# Autodesk Inventor assembly: SPE0V1 Ensamble General
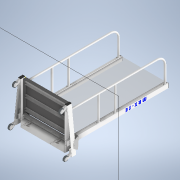
[picture p0: Inventor's stored thumbnail of the model, 180x180]
Saved by Autodesk Inventor 2021.2 (Build 252289000, 289)
## iProperties
Created: 2026-05-12
Part Number: SPE0V1 Ensamble General
Document SubType Name: Assembly
Designer: nelso
Author: nelso
## Documents named in this file (14)
- C:\Users\nelso\Desktop\Soporte-Paciente-Espinografia\Workspace\SPE0V1 Ensamble General.iam
- C:\Users\nelso\Desktop\Soporte-Paciente-Espinografia\Workspace\SP25V1 Acrilico.ipt
- C:\Users\nelso\Desktop\Soporte-Paciente-Espinografia\Workspace\SPE1V1 Estructura.iam
- C:\Users\nelso\Desktop\Soporte-Paciente-Espinografia\Workspace\SPE2V1 Baranda.iam
- C:\Users\nelso\Desktop\Soporte-Paciente-Espinografia\Workspace\DIN933M8X1.25L20C.ipt
- C:\Users\nelso\Desktop\Soporte-Paciente-Espinografia\Workspace\DIN125-A8,4C.ipt
- C:\Users\nelso\Desktop\Soporte-Paciente-Espinografia\Workspace\Logo.ipt
- C:\Users\nelso\Desktop\Soporte-Paciente-Espinografia\Workspace\SP28V1 Seguro Acrilico.ipt
- C:\Users\nelso\Desktop\Soporte-Paciente-Espinografia\Workspace\SP26V1 Base Chapa.ipt
- C:\Users\nelso\Desktop\Soporte-Paciente-Espinografia\Workspace\SP32V1 Refuerzo.ipt
- C:\Users\nelso\Desktop\Soporte-Paciente-Espinografia\Workspace\SPE31V1 Bisagra.iam
- C:\Users\nelso\Desktop\Soporte-Paciente-Espinografia\Workspace\SP39V1 Chapa Acrilico.ipt
- C:\Users\nelso\Desktop\Soporte-Paciente-Espinografia\Workspace\ISO7380M4X0.8L16I.ipt
- C:\Users\nelso\Desktop\Soporte-Paciente-Espinografia\Workspace\DIN555-5M4X0.8I.ipt
## Components (84 placed, 13 different names)
1. SP26V1 Base Chapa:1 — Mate:343, Mate:344, Mate:345, Mate:346, Mate:347, Mate:348, Mate:350, Mate:351, Mate:352, Mate:353, Mate:354, Flush:49, Flush:50, Flush:51, Angle:1
2. SP25V1 Acrilico:1 — Mate:179, Mate:180, Flush:19, Flush:20, Mate:262, Mate:355, Mate:356, Mate:357, Flush:52, Flush:53
3. SPE1V1 Estructura:1 [sub-assembly] — Coincidencia:100, Coincidencia:101, Coincidencia:102, Coincidencia:117, Nivelación:14, Nivelación:15, Mate:235, Mate:236, Mate:237, Flush:40, Mate:239, Mate:240, Mate:241, Flush:42, Mate:324, Mate:325, Flush:47, Flush:48, Mate:331, Mate:332, Mate:333, Mate:337, Mate:338, Mate:339, Mate:340, Mate:341, Mate:342, Angle:1, Flush:52
4. SPE2V1 Baranda:2 [sub-assembly] — Coincidencia:100, Coincidencia:101, Coincidencia:102, Coincidencia:109, Coincidencia:110, Coincidencia:111, Coincidencia:112, Mate:134, Mate:135, Mate:136, Mate:137, Mate:138, Mate:139, Mate:140, Mate:141, Mate:142, Mate:143, Mate:144, Mate:145, Mate:168, Mate:169, Mate:170, Mate:171, Mate:172, Mate:173
5. SPE2V1 Baranda:3 [sub-assembly] — Mate:118, Mate:119, Mate:120, Mate:121, Mate:122, Mate:123, Mate:124, Mate:125, Mate:126, Mate:127, Mate:128, Mate:129, Mate:130, Mate:131, Mate:132, Mate:133, Mate:147, Mate:149, Mate:156, Mate:157, Mate:158, Mate:159, Mate:160, Mate:161, Mate:235, Mate:236
6. DIN933M8X1.25L20C:1 — Coincidencia:113, Coincidencia:114
7. DIN125-A8,4C:1 — Coincidencia:109, Coincidencia:110, Coincidencia:115, Coincidencia:116
8. DIN125-A8,4C:2 — Coincidencia:111, Coincidencia:112, Coincidencia:113, Coincidencia:114
9. DIN933M8X1.25L20C:2 — Coincidencia:115, Coincidencia:116
10. Logo:1 — Coincidencia:117, Nivelación:14, Nivelación:15
11. DIN125-A8,4C:3 — Mate:144, Mate:145, Mate:162
12. DIN125-A8,4C:4 — Mate:142, Mate:143, Mate:163
13. DIN125-A8,4C:5 — Mate:140, Mate:141, Mate:164
14. DIN125-A8,4C:6 — Mate:138, Mate:139, Mate:165
15. DIN125-A8,4C:7 — Mate:135, Mate:136, Mate:167
16. DIN125-A8,4C:8 — Mate:134, Mate:137, Mate:166
17. DIN125-A8,4C:9 — Mate:130, Mate:132, Mate:155
18. DIN125-A8,4C:10 — Mate:131, Mate:133, Mate:154
19. DIN125-A8,4C:11 — Mate:128, Mate:129, Mate:153
20. DIN125-A8,4C:12 — Mate:126, Mate:127, Mate:152
21. DIN125-A8,4C:13 — Mate:122, Mate:123, Mate:150
22. DIN125-A8,4C:14 — Mate:124, Mate:125, Mate:151
23. DIN125-A8,4C:15 — Mate:120, Mate:121, Mate:148
24. DIN125-A8,4C:16 — Mate:118, Mate:119, Mate:146
25. DIN933M8X1.25L20C:3 — Mate:162, Mate:168
26. DIN933M8X1.25L20C:4 — Mate:163, Mate:169
27. DIN933M8X1.25L20C:5 — Mate:164, Mate:170
28. DIN933M8X1.25L20C:6 — Mate:165, Mate:171
29. DIN933M8X1.25L20C:7 — Mate:166, Mate:172
30. DIN933M8X1.25L20C:8 — Mate:167, Mate:173
31. DIN933M8X1.25L20C:9 — Mate:155, Mate:156
32. DIN933M8X1.25L20C:10 — Mate:154, Mate:157
33. DIN933M8X1.25L20C:11 — Mate:153, Mate:159
34. DIN933M8X1.25L20C:12 — Mate:152, Mate:158
35. DIN933M8X1.25L20C:13 — Mate:151, Mate:160
36. DIN933M8X1.25L20C:14 — Mate:150, Mate:161, Mate:237
37. DIN933M8X1.25L20C:15 — Mate:148, Mate:149
38. DIN933M8X1.25L20C:16 — Mate:146, Mate:147
39. SP28V1 Seguro Acrilico:1 — Mate:179, Flush:19, Mate:199, Mate:200, Mate:201, Mate:202, Mate:203, Mate:204, Mate:205, Mate:206, Mate:207, Mate:217, Mate:218, Mate:219, Mate:220, Mate:221, Mate:222, Mate:223, Mate:224, Mate:225, Flush:53
40. SP28V1 Seguro Acrilico:2 — Mate:180, Flush:20, Mate:208, Mate:209, Mate:210, Mate:211, Mate:212, Mate:213, Mate:214, Mate:215, Mate:216, Mate:226, Mate:227, Mate:228, Mate:229, Mate:230, Mate:231, Mate:232, Mate:233, Mate:234, Flush:40, Flush:42
41. ISO7380M4X0.8L16I:1 — Mate:199, Mate:217, Mate:358
42. ISO7380M4X0.8L16I:2 — Mate:200, Mate:218, Mate:359
43. ISO7380M4X0.8L16I:3 — Mate:201, Mate:219, Mate:360
44. ISO7380M4X0.8L16I:4 — Mate:202, Mate:220, Mate:361
45. ISO7380M4X0.8L16I:5 — Mate:203, Mate:221, Mate:362
46. ISO7380M4X0.8L16I:6 — Mate:204, Mate:222, Mate:363
47. ISO7380M4X0.8L16I:7 — Mate:205, Mate:223, Mate:364
48. ISO7380M4X0.8L16I:8 — Mate:206, Mate:224, Mate:365
49. ISO7380M4X0.8L16I:9 — Mate:207, Mate:225, Mate:366
50. ISO7380M4X0.8L16I:10 — Mate:208, Mate:234, Mate:262, Mate:367
51. ISO7380M4X0.8L16I:11 — Mate:209, Mate:233, Mate:368
52. ISO7380M4X0.8L16I:12 — Mate:210, Mate:232, Mate:369
53. ISO7380M4X0.8L16I:13 — Mate:211, Mate:231, Mate:370
54. ISO7380M4X0.8L16I:14 — Mate:212, Mate:230, Mate:371
55. ISO7380M4X0.8L16I:15 — Mate:214, Mate:228, Mate:373
56. ISO7380M4X0.8L16I:16 — Mate:215, Mate:227, Mate:374
57. ISO7380M4X0.8L16I:17 — Mate:216, Mate:226, Mate:375
58. ISO7380M4X0.8L16I:18 — Mate:213, Mate:229, Mate:372
59. SP32V1 Refuerzo:1 — Mate:351, Mate:354, Flush:50
60. SP32V1 Refuerzo:2 — Mate:348, Mate:353, Flush:49
61. SP32V1 Refuerzo:3 — Mate:350, Mate:352, Flush:51
62. SPE31V1 Bisagra:1 [sub-assembly] — Mate:333, Mate:341, Mate:342, Mate:345, Mate:347
63. SPE31V1 Bisagra:2 [sub-assembly] — Mate:331, Mate:337, Mate:338, Mate:344, Mate:346
64. SPE31V1 Bisagra:3 [sub-assembly] — Mate:332, Mate:339, Mate:340, Mate:343
65. SP39V1 Chapa Acrilico:1 — Mate:325, Flush:47, Mate:355, Mate:380, Mate:381, Mate:382, Mate:383, Mate:384, Mate:385, Mate:386, Mate:387, Mate:388
66. SP39V1 Chapa Acrilico:2 — Mate:324, Flush:48, Mate:357, Mate:376, Mate:377, Mate:378, Mate:379, Mate:389, Mate:390, Mate:391, Mate:392, Mate:393
67. DIN555-5M4X0.8I:1 — Mate:358, Mate:376
68. DIN555-5M4X0.8I:2 — Mate:359, Mate:377
69. DIN555-5M4X0.8I:3 — Mate:360, Mate:378
70. DIN555-5M4X0.8I:4 — Mate:361, Mate:379
71. DIN555-5M4X0.8I:5 — Mate:362, Mate:389
72. DIN555-5M4X0.8I:6 — Mate:363, Mate:390
73. DIN555-5M4X0.8I:7 — Mate:364, Mate:391
74. DIN555-5M4X0.8I:8 — Mate:365, Mate:392
75. DIN555-5M4X0.8I:9 — Mate:366, Mate:393
76. DIN555-5M4X0.8I:10 — Mate:367, Mate:380
77. DIN555-5M4X0.8I:11 — Mate:368, Mate:381
78. DIN555-5M4X0.8I:12 — Mate:369, Mate:382
79. DIN555-5M4X0.8I:13 — Mate:370, Mate:383
80. DIN555-5M4X0.8I:14 — Mate:371, Mate:384
81. DIN555-5M4X0.8I:15 — Mate:372, Mate:385
82. DIN555-5M4X0.8I:16 — Mate:373, Mate:386
83. DIN555-5M4X0.8I:17 — Mate:374, Mate:387
84. DIN555-5M4X0.8I:18 — Mate:375, Mate:388
## Relationships (188: Mate 174, Flush 13, Angle 1)
- Coincidencia:100 [Mate]: SPE1V1 Estructura:1 ↔ SPE2V1 Baranda:2
- Coincidencia:101 [Mate]: SPE1V1 Estructura:1 ↔ SPE2V1 Baranda:2
- Coincidencia:102 [Mate]: SPE1V1 Estructura:1 ↔ SPE2V1 Baranda:2
- Coincidencia:109 [Mate]: SPE2V1 Baranda:2 ↔ DIN125-A8,4C:1
- Coincidencia:110 [Mate]: SPE2V1 Baranda:2 ↔ DIN125-A8,4C:1
- Coincidencia:111 [Mate]: SPE2V1 Baranda:2 ↔ DIN125-A8,4C:2
- Coincidencia:112 [Mate]: SPE2V1 Baranda:2 ↔ DIN125-A8,4C:2
- Coincidencia:113 [Mate]: DIN933M8X1.25L20C:1 ↔ DIN125-A8,4C:2
- Coincidencia:114 [Mate]: DIN933M8X1.25L20C:1 ↔ DIN125-A8,4C:2
- Coincidencia:115 [Mate]: DIN125-A8,4C:1 ↔ DIN933M8X1.25L20C:2
- Coincidencia:116 [Mate]: DIN125-A8,4C:1 ↔ DIN933M8X1.25L20C:2
- Coincidencia:117 [Mate]: SPE1V1 Estructura:1 ↔ Logo:1
- Nivelación:14 [Flush] (10 mm): SPE1V1 Estructura:1 ↔ Logo:1
- Nivelación:15 [Flush] (400 mm): SPE1V1 Estructura:1 ↔ Logo:1
- Mate:118: SPE2V1 Baranda:3 ↔ DIN125-A8,4C:16
- Mate:119: SPE2V1 Baranda:3 ↔ DIN125-A8,4C:16
- Mate:120: SPE2V1 Baranda:3 ↔ DIN125-A8,4C:15
- Mate:121: SPE2V1 Baranda:3 ↔ DIN125-A8,4C:15
- Mate:122: SPE2V1 Baranda:3 ↔ DIN125-A8,4C:13
- Mate:123: SPE2V1 Baranda:3 ↔ DIN125-A8,4C:13
- Mate:124: SPE2V1 Baranda:3 ↔ DIN125-A8,4C:14
- Mate:125: SPE2V1 Baranda:3 ↔ DIN125-A8,4C:14
- Mate:126: SPE2V1 Baranda:3 ↔ DIN125-A8,4C:12
- Mate:127: SPE2V1 Baranda:3 ↔ DIN125-A8,4C:12
- Mate:128: SPE2V1 Baranda:3 ↔ DIN125-A8,4C:11
- Mate:129: SPE2V1 Baranda:3 ↔ DIN125-A8,4C:11
- Mate:130: SPE2V1 Baranda:3 ↔ DIN125-A8,4C:9
- Mate:131: SPE2V1 Baranda:3 ↔ DIN125-A8,4C:10
- Mate:132: SPE2V1 Baranda:3 ↔ DIN125-A8,4C:9
- Mate:133: SPE2V1 Baranda:3 ↔ DIN125-A8,4C:10
- Mate:134: SPE2V1 Baranda:2 ↔ DIN125-A8,4C:8
- Mate:135: SPE2V1 Baranda:2 ↔ DIN125-A8,4C:7
- Mate:136: SPE2V1 Baranda:2 ↔ DIN125-A8,4C:7
- Mate:137: SPE2V1 Baranda:2 ↔ DIN125-A8,4C:8
- Mate:138: SPE2V1 Baranda:2 ↔ DIN125-A8,4C:6
- Mate:139: SPE2V1 Baranda:2 ↔ DIN125-A8,4C:6
- Mate:140: SPE2V1 Baranda:2 ↔ DIN125-A8,4C:5
- Mate:141: SPE2V1 Baranda:2 ↔ DIN125-A8,4C:5
- Mate:142: SPE2V1 Baranda:2 ↔ DIN125-A8,4C:4
- Mate:143: SPE2V1 Baranda:2 ↔ DIN125-A8,4C:4
- Mate:144: SPE2V1 Baranda:2 ↔ DIN125-A8,4C:3
- Mate:145: SPE2V1 Baranda:2 ↔ DIN125-A8,4C:3
- Mate:146: DIN125-A8,4C:16 ↔ DIN933M8X1.25L20C:16
- Mate:147: SPE2V1 Baranda:3 ↔ DIN933M8X1.25L20C:16
- Mate:148: DIN125-A8,4C:15 ↔ DIN933M8X1.25L20C:15
- Mate:149: SPE2V1 Baranda:3 ↔ DIN933M8X1.25L20C:15
- Mate:150: DIN125-A8,4C:13 ↔ DIN933M8X1.25L20C:14
- Mate:151: DIN125-A8,4C:14 ↔ DIN933M8X1.25L20C:13
- Mate:152: DIN125-A8,4C:12 ↔ DIN933M8X1.25L20C:12
- Mate:153: DIN125-A8,4C:11 ↔ DIN933M8X1.25L20C:11
- Mate:154: DIN125-A8,4C:10 ↔ DIN933M8X1.25L20C:10
- Mate:155: DIN125-A8,4C:9 ↔ DIN933M8X1.25L20C:9
- Mate:156: SPE2V1 Baranda:3 ↔ DIN933M8X1.25L20C:9
- Mate:157: SPE2V1 Baranda:3 ↔ DIN933M8X1.25L20C:10
- Mate:158: SPE2V1 Baranda:3 ↔ DIN933M8X1.25L20C:12
- Mate:159: SPE2V1 Baranda:3 ↔ DIN933M8X1.25L20C:11
- Mate:160: SPE2V1 Baranda:3 ↔ DIN933M8X1.25L20C:13
- Mate:161: SPE2V1 Baranda:3 ↔ DIN933M8X1.25L20C:14
- Mate:162: DIN125-A8,4C:3 ↔ DIN933M8X1.25L20C:3
- Mate:163: DIN125-A8,4C:4 ↔ DIN933M8X1.25L20C:4
- Mate:164: DIN125-A8,4C:5 ↔ DIN933M8X1.25L20C:5
- Mate:165: DIN125-A8,4C:6 ↔ DIN933M8X1.25L20C:6
- Mate:166: DIN125-A8,4C:8 ↔ DIN933M8X1.25L20C:7
- Mate:167: DIN125-A8,4C:7 ↔ DIN933M8X1.25L20C:8
- Mate:168: SPE2V1 Baranda:2 ↔ DIN933M8X1.25L20C:3
- Mate:169: SPE2V1 Baranda:2 ↔ DIN933M8X1.25L20C:4
- Mate:170: SPE2V1 Baranda:2 ↔ DIN933M8X1.25L20C:5
- Mate:171: SPE2V1 Baranda:2 ↔ DIN933M8X1.25L20C:6
- Mate:172: SPE2V1 Baranda:2 ↔ DIN933M8X1.25L20C:7
- Mate:173: SPE2V1 Baranda:2 ↔ DIN933M8X1.25L20C:8
- Mate:179: SP25V1 Acrilico:1 ↔ SP28V1 Seguro Acrilico:1
- Mate:180: SP25V1 Acrilico:1 ↔ SP28V1 Seguro Acrilico:2
- Flush:19: SP25V1 Acrilico:1 ↔ SP28V1 Seguro Acrilico:1
- Flush:20: SP25V1 Acrilico:1 ↔ SP28V1 Seguro Acrilico:2
- Mate:199: SP28V1 Seguro Acrilico:1 ↔ ISO7380M4X0.8L16I:1
- Mate:200: SP28V1 Seguro Acrilico:1 ↔ ISO7380M4X0.8L16I:2
- Mate:201: SP28V1 Seguro Acrilico:1 ↔ ISO7380M4X0.8L16I:3
- Mate:202: SP28V1 Seguro Acrilico:1 ↔ ISO7380M4X0.8L16I:4
- Mate:203: SP28V1 Seguro Acrilico:1 ↔ ISO7380M4X0.8L16I:5
- Mate:204: SP28V1 Seguro Acrilico:1 ↔ ISO7380M4X0.8L16I:6
- Mate:205: SP28V1 Seguro Acrilico:1 ↔ ISO7380M4X0.8L16I:7
- Mate:206: SP28V1 Seguro Acrilico:1 ↔ ISO7380M4X0.8L16I:8
- Mate:207: SP28V1 Seguro Acrilico:1 ↔ ISO7380M4X0.8L16I:9
- Mate:208: SP28V1 Seguro Acrilico:2 ↔ ISO7380M4X0.8L16I:10
- Mate:209: SP28V1 Seguro Acrilico:2 ↔ ISO7380M4X0.8L16I:11
- Mate:210: SP28V1 Seguro Acrilico:2 ↔ ISO7380M4X0.8L16I:12
- Mate:211: SP28V1 Seguro Acrilico:2 ↔ ISO7380M4X0.8L16I:13
- Mate:212: SP28V1 Seguro Acrilico:2 ↔ ISO7380M4X0.8L16I:14
- Mate:213: SP28V1 Seguro Acrilico:2 ↔ ISO7380M4X0.8L16I:18
- Mate:214: SP28V1 Seguro Acrilico:2 ↔ ISO7380M4X0.8L16I:15
- Mate:215: SP28V1 Seguro Acrilico:2 ↔ ISO7380M4X0.8L16I:16
- Mate:216: SP28V1 Seguro Acrilico:2 ↔ ISO7380M4X0.8L16I:17
- Mate:217: SP28V1 Seguro Acrilico:1 ↔ ISO7380M4X0.8L16I:1
- Mate:218: SP28V1 Seguro Acrilico:1 ↔ ISO7380M4X0.8L16I:2
- Mate:219: SP28V1 Seguro Acrilico:1 ↔ ISO7380M4X0.8L16I:3
- Mate:220: SP28V1 Seguro Acrilico:1 ↔ ISO7380M4X0.8L16I:4
- Mate:221: SP28V1 Seguro Acrilico:1 ↔ ISO7380M4X0.8L16I:5
- Mate:222: SP28V1 Seguro Acrilico:1 ↔ ISO7380M4X0.8L16I:6
- Mate:223: SP28V1 Seguro Acrilico:1 ↔ ISO7380M4X0.8L16I:7
- Mate:224: SP28V1 Seguro Acrilico:1 ↔ ISO7380M4X0.8L16I:8
- Mate:225: SP28V1 Seguro Acrilico:1 ↔ ISO7380M4X0.8L16I:9
- Mate:226: SP28V1 Seguro Acrilico:2 ↔ ISO7380M4X0.8L16I:17
- Mate:227: SP28V1 Seguro Acrilico:2 ↔ ISO7380M4X0.8L16I:16
- Mate:228: SP28V1 Seguro Acrilico:2 ↔ ISO7380M4X0.8L16I:15
- Mate:229: SP28V1 Seguro Acrilico:2 ↔ ISO7380M4X0.8L16I:18
- Mate:230: SP28V1 Seguro Acrilico:2 ↔ ISO7380M4X0.8L16I:14
- Mate:231: SP28V1 Seguro Acrilico:2 ↔ ISO7380M4X0.8L16I:13
- Mate:232: SP28V1 Seguro Acrilico:2 ↔ ISO7380M4X0.8L16I:12
- Mate:233: SP28V1 Seguro Acrilico:2 ↔ ISO7380M4X0.8L16I:11
- Mate:234: SP28V1 Seguro Acrilico:2 ↔ ISO7380M4X0.8L16I:10
- Mate:235: SPE1V1 Estructura:1 ↔ SPE2V1 Baranda:3
- Mate:236: SPE1V1 Estructura:1 ↔ SPE2V1 Baranda:3
- Mate:237: SPE1V1 Estructura:1 ↔ DIN933M8X1.25L20C:14
- Flush:40: SPE1V1 Estructura:1 ↔ SP28V1 Seguro Acrilico:2
- Mate:239: SPE1V1 Estructura:1
- Mate:240: SPE1V1 Estructura:1
- Mate:241: SPE1V1 Estructura:1
- Flush:42: SPE1V1 Estructura:1 ↔ SP28V1 Seguro Acrilico:2
- Mate:262: SP25V1 Acrilico:1 ↔ ISO7380M4X0.8L16I:10
- Mate:324: SPE1V1 Estructura:1 ↔ SP39V1 Chapa Acrilico:2
- Mate:325: SPE1V1 Estructura:1 ↔ SP39V1 Chapa Acrilico:1
- Flush:47: SPE1V1 Estructura:1 ↔ SP39V1 Chapa Acrilico:1
- Flush:48: SPE1V1 Estructura:1 ↔ SP39V1 Chapa Acrilico:2
- Mate:331: SPE1V1 Estructura:1 ↔ SPE31V1 Bisagra:2
- Mate:332: SPE1V1 Estructura:1 ↔ SPE31V1 Bisagra:3
- Mate:333: SPE1V1 Estructura:1 ↔ SPE31V1 Bisagra:1
- Mate:337: SPE1V1 Estructura:1 ↔ SPE31V1 Bisagra:2
- Mate:338: SPE1V1 Estructura:1 ↔ SPE31V1 Bisagra:2
- Mate:339: SPE1V1 Estructura:1 ↔ SPE31V1 Bisagra:3
- Mate:340: SPE1V1 Estructura:1 ↔ SPE31V1 Bisagra:3
- Mate:341: SPE1V1 Estructura:1 ↔ SPE31V1 Bisagra:1
- Mate:342: SPE1V1 Estructura:1 ↔ SPE31V1 Bisagra:1
- Mate:343: SP26V1 Base Chapa:1 ↔ SPE31V1 Bisagra:3
- Mate:344: SP26V1 Base Chapa:1 ↔ SPE31V1 Bisagra:2
- Mate:345: SP26V1 Base Chapa:1 ↔ SPE31V1 Bisagra:1
- Mate:346: SP26V1 Base Chapa:1 ↔ SPE31V1 Bisagra:2
- Mate:347: SP26V1 Base Chapa:1 ↔ SPE31V1 Bisagra:1
- Mate:348: SP26V1 Base Chapa:1 ↔ SP32V1 Refuerzo:2
- Mate:350: SP26V1 Base Chapa:1 ↔ SP32V1 Refuerzo:3
- Mate:351: SP26V1 Base Chapa:1 ↔ SP32V1 Refuerzo:1
- Mate:352: SP26V1 Base Chapa:1 ↔ SP32V1 Refuerzo:3
- Mate:353: SP26V1 Base Chapa:1 ↔ SP32V1 Refuerzo:2
- Mate:354: SP26V1 Base Chapa:1 ↔ SP32V1 Refuerzo:1
- Flush:49: SP26V1 Base Chapa:1 ↔ SP32V1 Refuerzo:2
- Flush:50: SP26V1 Base Chapa:1 ↔ SP32V1 Refuerzo:1
- Flush:51: SP26V1 Base Chapa:1 ↔ SP32V1 Refuerzo:3
- Angle:1 (0 deg): SP26V1 Base Chapa:1 ↔ SPE1V1 Estructura:1
- Mate:355: SP25V1 Acrilico:1 ↔ SP39V1 Chapa Acrilico:1
- Mate:356: SP25V1 Acrilico:1
- Mate:357: SP25V1 Acrilico:1 ↔ SP39V1 Chapa Acrilico:2
- Flush:52: SP25V1 Acrilico:1 ↔ SPE1V1 Estructura:1
- Flush:53: SP25V1 Acrilico:1 ↔ SP28V1 Seguro Acrilico:1
- Mate:358: ISO7380M4X0.8L16I:1 ↔ DIN555-5M4X0.8I:1
- Mate:359: ISO7380M4X0.8L16I:2 ↔ DIN555-5M4X0.8I:2
- Mate:360: ISO7380M4X0.8L16I:3 ↔ DIN555-5M4X0.8I:3
- Mate:361: ISO7380M4X0.8L16I:4 ↔ DIN555-5M4X0.8I:4
- Mate:362: ISO7380M4X0.8L16I:5 ↔ DIN555-5M4X0.8I:5
- Mate:363: ISO7380M4X0.8L16I:6 ↔ DIN555-5M4X0.8I:6
- Mate:364: ISO7380M4X0.8L16I:7 ↔ DIN555-5M4X0.8I:7
- Mate:365: ISO7380M4X0.8L16I:8 ↔ DIN555-5M4X0.8I:8
- Mate:366: ISO7380M4X0.8L16I:9 ↔ DIN555-5M4X0.8I:9
- Mate:367: ISO7380M4X0.8L16I:10 ↔ DIN555-5M4X0.8I:10
- Mate:368: ISO7380M4X0.8L16I:11 ↔ DIN555-5M4X0.8I:11
- Mate:369: ISO7380M4X0.8L16I:12 ↔ DIN555-5M4X0.8I:12
- Mate:370: ISO7380M4X0.8L16I:13 ↔ DIN555-5M4X0.8I:13
- Mate:371: ISO7380M4X0.8L16I:14 ↔ DIN555-5M4X0.8I:14
- Mate:372: ISO7380M4X0.8L16I:18 ↔ DIN555-5M4X0.8I:15
- Mate:373: ISO7380M4X0.8L16I:15 ↔ DIN555-5M4X0.8I:16
- Mate:374: ISO7380M4X0.8L16I:16 ↔ DIN555-5M4X0.8I:17
- Mate:375: ISO7380M4X0.8L16I:17 ↔ DIN555-5M4X0.8I:18
- Mate:376: SP39V1 Chapa Acrilico:2 ↔ DIN555-5M4X0.8I:1
- Mate:377: SP39V1 Chapa Acrilico:2 ↔ DIN555-5M4X0.8I:2
- Mate:378: SP39V1 Chapa Acrilico:2 ↔ DIN555-5M4X0.8I:3
- Mate:379: SP39V1 Chapa Acrilico:2 ↔ DIN555-5M4X0.8I:4
- Mate:380: SP39V1 Chapa Acrilico:1 ↔ DIN555-5M4X0.8I:10
- Mate:381: SP39V1 Chapa Acrilico:1 ↔ DIN555-5M4X0.8I:11
- Mate:382: SP39V1 Chapa Acrilico:1 ↔ DIN555-5M4X0.8I:12
- Mate:383: SP39V1 Chapa Acrilico:1 ↔ DIN555-5M4X0.8I:13
- Mate:384: SP39V1 Chapa Acrilico:1 ↔ DIN555-5M4X0.8I:14
- Mate:385: SP39V1 Chapa Acrilico:1 ↔ DIN555-5M4X0.8I:15
- Mate:386: SP39V1 Chapa Acrilico:1 ↔ DIN555-5M4X0.8I:16
- Mate:387: SP39V1 Chapa Acrilico:1 ↔ DIN555-5M4X0.8I:17
- Mate:388: SP39V1 Chapa Acrilico:1 ↔ DIN555-5M4X0.8I:18
- Mate:389: SP39V1 Chapa Acrilico:2 ↔ DIN555-5M4X0.8I:5
- Mate:390: SP39V1 Chapa Acrilico:2 ↔ DIN555-5M4X0.8I:6
- Mate:391: SP39V1 Chapa Acrilico:2 ↔ DIN555-5M4X0.8I:7
- Mate:392: SP39V1 Chapa Acrilico:2 ↔ DIN555-5M4X0.8I:8
- Mate:393: SP39V1 Chapa Acrilico:2 ↔ DIN555-5M4X0.8I:9
